# Autodesk Inventor assembly: Ensamble
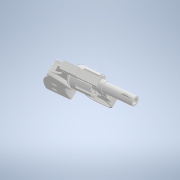
[picture p0: Inventor's stored thumbnail of the model, 180x180]
Saved by Autodesk Inventor 2021 (Build 250183000, 183)
## iProperties
Created: 2022-03-10
Part Number: Ensamble
Document SubType Name: Assembly
Designer: Carlos Montoya
Author: Carlos Montoya
## Documents named in this file (10)
- D:\TEC\Semestre 12\Manufactura\hechos\Ensamble.iam
- D:\TEC\Semestre 12\Manufactura\hechos\Telo_Levo_1.ipt
- D:\TEC\Semestre 12\Manufactura\hechos\Telo_Desno_3.ipt
- D:\TEC\Semestre 12\Manufactura\hechos\Rukohvat_Levi_2.ipt
- D:\TEC\Semestre 12\Manufactura\hechos\Rukohvat_Desni_4.ipt
- D:\TEC\Semestre 12\Manufactura\hechos\Parte superior pistola.ipt
- D:\TEC\Semestre 12\Manufactura\hechos\Part2.ipt
- D:\TEC\Semestre 12\Manufactura\hechos\Fiksator.ipt
- D:\TEC\Semestre 12\Manufactura\hechos\Rucica.ipt
- D:\TEC\Semestre 12\Manufactura\hechos\Oruga_9.ipt
## Components (9 placed, 9 different names)
1. Telo_Levo_1:1 — Flush:1, Flush:2, Mate:1, Tangent:1, Tangent:2, Mate:2, Mate:9
2. Telo_Desno_3:1 — Flush:1, Flush:2, Mate:1, Mate:3, Mate:4, Mate:5, Mate:6, Mate:7
3. Rukohvat_Levi_2:1 — Tangent:1, Tangent:2, Mate:2
4. Rukohvat_Desni_4:1 — Mate:3, Mate:4, Mate:5
5. Parte superior pistola:1 — Mate:6, Mate:7, Mate:8, Mate:10, Mate:11
6. Part2:1 — Mate:8
7. Fiksator:1 — Mate:9, Mate:10
8. Rucica:1 — Mate:11
9. Oruga_9:1
## Relationships (15: Mate 11, Flush 2, Tangent 2)
- Flush:1: Telo_Levo_1:1 ↔ Telo_Desno_3:1
- Flush:2: Telo_Levo_1:1 ↔ Telo_Desno_3:1
- Mate:1: Telo_Levo_1:1 ↔ Telo_Desno_3:1
- Tangent:1: Telo_Levo_1:1 ↔ Rukohvat_Levi_2:1
- Tangent:2: Telo_Levo_1:1 ↔ Rukohvat_Levi_2:1
- Mate:2: Telo_Levo_1:1 ↔ Rukohvat_Levi_2:1
- Mate:3: Telo_Desno_3:1 ↔ Rukohvat_Desni_4:1
- Mate:4: Telo_Desno_3:1 ↔ Rukohvat_Desni_4:1
- Mate:5: Telo_Desno_3:1 ↔ Rukohvat_Desni_4:1
- Mate:6: Telo_Desno_3:1 ↔ Parte superior pistola:1
- Mate:7: Telo_Desno_3:1 ↔ Parte superior pistola:1
- Mate:8: Parte superior pistola:1 ↔ Part2:1
- Mate:9: Telo_Levo_1:1 ↔ Fiksator:1
- Mate:10: Parte superior pistola:1 ↔ Fiksator:1
- Mate:11: Parte superior pistola:1 ↔ Rucica:1
